# Autodesk Inventor assembly: Avionics
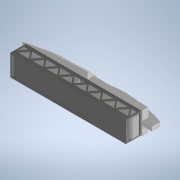
[picture p0: Inventor's stored thumbnail of the model, 180x180]
Saved by Autodesk Inventor 2020.4 (Build 244396000, 396)
## iProperties
Created: 2021-04-27
Part Number: Avionics
Document SubType Name: Assembly
Designer: armin
Author: armin
## Documents named in this file (4)
- C:\Users\armin\Documents\Inventor 3D filer\Flyver\Avionics.iam
- C:\Users\armin\Documents\Inventor 3D filer\Flyver\Avionics\AvionicsLit.ipt
- C:\Users\armin\Documents\Inventor 3D filer\Flyver\LiPo.ipt
- C:\Users\armin\Documents\Inventor 3D filer\Flyver\Avionics\Avionics frame.ipt
## Components (4 placed, 3 different names)
1. AvionicsLit:1 — Mate:2, Flush:3, Flush:4
2. LiPo:1 — Flush:1, Mate:1, Flush:2
3. LiPo:2 — Flush:1, Mate:1, Flush:2, Mate:3, Mate:4
4. Avionics frame:1 — Mate:2, Flush:3, Flush:4, Mate:3, Mate:4
## Relationships (8: Flush 4, Mate 4)
- Flush:1: LiPo:1 ↔ LiPo:2
- Mate:1 (2 mm): LiPo:1 ↔ LiPo:2
- Flush:2: LiPo:1 ↔ LiPo:2
- Mate:2: AvionicsLit:1 ↔ Avionics frame:1
- Flush:3 (1 mm): AvionicsLit:1 ↔ Avionics frame:1
- Flush:4 (2 mm): AvionicsLit:1 ↔ Avionics frame:1
- Mate:3 (0.5 mm): LiPo:2 ↔ Avionics frame:1
- Mate:4: LiPo:2 ↔ Avionics frame:1
